# Autodesk Inventor assembly: draft assembly 2
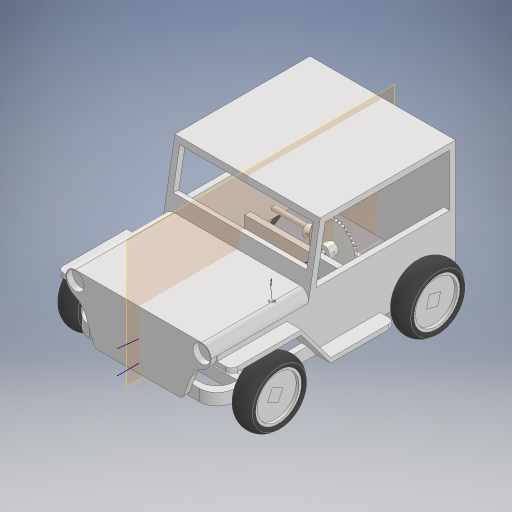
[picture p0: Inventor's stored thumbnail of the model, 512x512]
Saved by Autodesk Inventor 2024 (Build 280153000, 153)
## iProperties
Created: 2024-04-13
Part Number: draft assembly 2
Document SubType Name: Assembly
Designer: Alex
Author: Alex
## Documents named in this file (7)
- C:\Shared\alex-bartella-schoolwork\4z03\final\draft assembly 2.iam
- C:\Shared\alex-bartella-schoolwork\4z03\final\shell.ipt
- C:\Shared\alex-bartella-schoolwork\4z03\final\front axle.ipt
- C:\Shared\alex-bartella-schoolwork\4z03\final\final\wheel.iam
- C:\Shared\alex-bartella-schoolwork\4z03\final\rear axle.ipt
- C:\Shared\alex-bartella-schoolwork\4z03\final\rc_motor\rc_motor.ipt
- C:\Shared\alex-bartella-schoolwork\4z03\final\final\gears\Bevel Gears4.iam
## Components (9 placed, 6 different names)
1. shell:1 — Flush:1, Flush:2, Flush:3, Mate:1, Mate:4, Mate:7, Mate:10, Mate:16, Angle:2, Mate:18, Angle:3, Mate:19, Angle:4
2. front axle:1 — Mate:1, Mate:2, Mate:3, Mate:5, Mate:6
3. wheel:1 [sub-assembly] — Mate:2, Mate:3, Mate:4
4. wheel:2 [sub-assembly] — Mate:5, Mate:6
5. rear axle:1 — Mate:7, Mate:8, Mate:9, Mate:11, Mate:12
6. wheel:3 [sub-assembly] — Mate:8, Mate:9, Mate:10
7. wheel:4 [sub-assembly] — Mate:11, Mate:12
8. rc_motor:1 — Mate:16, Angle:2, Mate:17
9. Bevel Gears:1 [sub-assembly] — Mate:17
## Relationships (23: Mate 16, Flush 3, Angle 3, Symmetry 1)
- Flush:1: shell:1
- Flush:2: shell:1
- Flush:3: shell:1
- Mate:1: shell:1 ↔ front axle:1
- Mate:2: front axle:1 ↔ wheel:1
- Mate:3: front axle:1 ↔ wheel:1
- Mate:4: shell:1 ↔ wheel:1
- Mate:5: front axle:1 ↔ wheel:2
- Mate:6: front axle:1 ↔ wheel:2
- Mate:7: shell:1 ↔ rear axle:1
- Mate:8: rear axle:1 ↔ wheel:3
- Mate:9: rear axle:1 ↔ wheel:3
- Mate:10: shell:1 ↔ wheel:3
- Mate:11: rear axle:1 ↔ wheel:4
- Mate:12: rear axle:1 ↔ wheel:4
- Mate:16: shell:1 ↔ rc_motor:1
- Angle:2 (0 deg): shell:1 ↔ rc_motor:1
- Mate:17: rc_motor:1 ↔ Bevel Gears:1
- Mate:18: shell:1
- Angle:3 (0 deg): shell:1
- Mate:19: shell:1
- Angle:4 (0 deg): shell:1
- Symmetry:1
